# Autodesk Inventor assembly: Foot
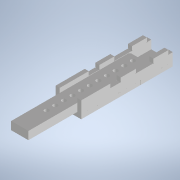
[picture p0: Inventor's stored thumbnail of the model, 180x180]
Saved by Autodesk Inventor 2020 (Build 240168000, 168)
## iProperties
Created: 2019-12-19
Part Number: Foot
Document SubType Name: Assembly
Designer: damien
Author: damien
## Documents named in this file (4)
- D:\fablab\sawbench\Foot.iam
- D:\fablab\sawbench\graduated_foot_03.ipt
- D:\fablab\sawbench\rail.ipt
- D:\fablab\sawbench\cover.ipt
## Components (5 placed, 3 different names)
1. graduated_foot_03:1 — Placage:1, Affleurement:1, Affleurement:2, Affleurement:3, Affleurement:4, Affleurement:5, Affleurement:6, Placage:6, Affleurement:8
2. graduated_foot_03:2 — Placage:1, Affleurement:1, Affleurement:2, Affleurement:3, Placage:12
3. rail:1 — Placage:6, Affleurement:8, Placage:9, Affleurement:9, Placage:10, Placage:11, Affleurement:11
4. cover:1 — Affleurement:10, Placage:11, Placage:12, Affleurement:11
5. cover:2 — Placage:9, Affleurement:9, Placage:10, Affleurement:10
## Relationships (16: Flush 10, Mate 6)
- Placage:1 [Mate]: graduated_foot_03:1 ↔ graduated_foot_03:2
- Affleurement:1 [Flush]: graduated_foot_03:1 ↔ graduated_foot_03:2
- Affleurement:2 [Flush]: graduated_foot_03:1 ↔ graduated_foot_03:2
- Affleurement:3 [Flush]: graduated_foot_03:1 ↔ graduated_foot_03:2
- Affleurement:4 [Flush]: graduated_foot_03:1
- Affleurement:5 [Flush]: graduated_foot_03:1
- Affleurement:6 [Flush]: graduated_foot_03:1
- Placage:6 [Mate]: graduated_foot_03:1 ↔ rail:1
- Affleurement:8 [Flush] (-100 mm): graduated_foot_03:1 ↔ rail:1
- Placage:9 [Mate]: rail:1 ↔ cover:2
- Affleurement:9 [Flush]: rail:1 ↔ cover:2
- Placage:10 [Mate]: rail:1 ↔ cover:2
- Affleurement:10 [Flush]: cover:1 ↔ cover:2
- Placage:11 [Mate]: rail:1 ↔ cover:1
- Placage:12 [Mate]: graduated_foot_03:2 ↔ cover:1
- Affleurement:11 [Flush]: rail:1 ↔ cover:1
